# Autodesk Inventor assembly: 전체 조립품
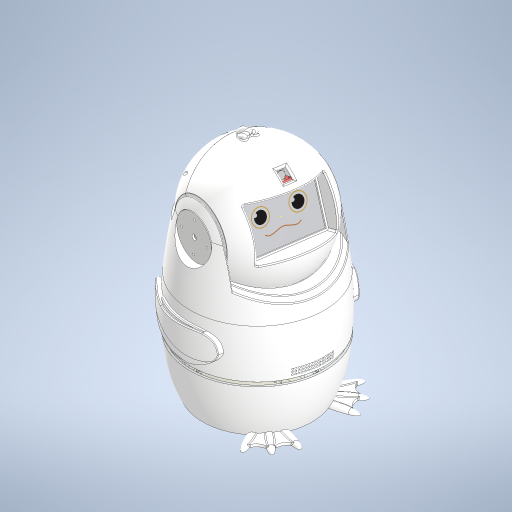
[picture p0: Inventor's stored thumbnail of the model, 512x512]
Saved by Autodesk Inventor 2023 (Build 270158000, 158)
## iProperties
Created: 2022-08-10
Part Number: 전체 조립품
Document SubType Name: Assembly
Designer: fly01
Author: fly01
## Documents named in this file (6)
- C:\Users\user\Desktop\PAI\PAI설계\조림품\전체 조립품.iam
- C:\Users\user\Desktop\PAI\PAI설계\조림품\머리 조립품.iam
- C:\Users\user\Desktop\PAI\PAI설계\출력품\우측 축.ipt
- C:\Users\user\Desktop\PAI\PAI설계\출력품\좌측 축.ipt
- C:\Users\user\Desktop\PAI\PAI설계\조림품\상단 조립품.iam
- C:\Users\user\Desktop\PAI\PAI설계\조림품\하단 조립품.iam
## Components (5 placed, 5 different names)
1. 머리 조립품:1 [sub-assembly] — 삽입:6
2. 우측 축:1 — 삽입:7
3. 좌측 축:1 — 삽입:8
4. 상단 조립품:1 [sub-assembly] — 삽입:6, 삽입:7, 삽입:8, 삽입:9
5. 하단 조립품:1 [sub-assembly] — 삽입:9
## Relationships (4: Insert 4)
- 삽입:6 [Insert]: 머리 조립품:1 ↔ 상단 조립품:1
- 삽입:7 [Insert]: 우측 축:1 ↔ 상단 조립품:1
- 삽입:8 [Insert]: 좌측 축:1 ↔ 상단 조립품:1
- 삽입:9 [Insert]: 상단 조립품:1 ↔ 하단 조립품:1
